# Autodesk Inventor assembly: rovPrototype3
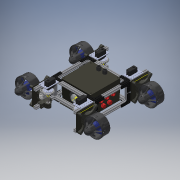
[picture p0: Inventor's stored thumbnail of the model, 180x180]
Saved by Autodesk Inventor 2018 (Build 220112000, 112)
## iProperties
Created: 2019-02-16
Part Number: rovPrototype3
Document SubType Name: Assembly
Designer: anirudh
Author: anirudh
## Documents named in this file (17)
- C:\Users\anirudh\Documents\MARS Fund\MATE Robotics\Silicon Sharks\2018-2019\Prototype3\rovPrototype3.iam
- C:\Users\anirudh\Documents\MARS Fund\MATE Robotics\Silicon Sharks\2018-2019\Prototype3\15inREV(3).ipt
- C:\Users\anirudh\Documents\MARS Fund\MATE Robotics\Silicon Sharks\2018-2019\Prototype3\LazySusanBearing(3).ipt
- C:\Users\anirudh\Documents\MARS Fund\Random CAD Files\REV-41-1305.ipt
- C:\Users\anirudh\Documents\MARS Fund\MATE Robotics\Silicon Sharks\2018-2019\Prototype3\12inREV(3).ipt
- C:\Users\anirudh\Documents\MARS Fund\MATE Robotics\Silicon Sharks\2018-2019\Prototype3\ThrusterMountv2(3).ipt
- C:\Users\anirudh\Documents\MARS Fund\MATE Robotics\Silicon Sharks\2018-2019\Prototype3\BevelGearTest(3).iam
- C:\Users\anirudh\Documents\MARS Fund\Random CAD Files\REV-41-1363.ipt
- C:\Users\anirudh\Documents\MARS Fund\MATE Robotics\Silicon Sharks\2018-2019\Prototype3\Servo(3).ipt
- C:\Users\anirudh\Documents\MARS Fund\Random CAD Files\REV-41-1028.ipt
- C:\Users\anirudh\Documents\MARS Fund\MATE Robotics\Silicon Sharks\2018-2019\Prototype3\4inREV(3).ipt
- C:\Users\anirudh\Documents\MARS Fund\MATE Robotics\Silicon Sharks\2018-2019\Prototype3\T200-THRUSTER(3).ipt
- C:\Users\anirudh\Documents\MARS Fund\MATE Robotics\Silicon Sharks\2018-2019\Prototype3\6mm-2.75inAxle(3).ipt
- C:\Users\anirudh\Documents\MARS Fund\MATE Robotics\Silicon Sharks\2018-2019\Prototype3\AxleBracket(3).ipt
- C:\Users\anirudh\Documents\MARS Fund\Random CAD Files\am-3377 6x12x4 Flanged Bearing.ipt
- C:\Users\anirudh\Documents\MARS Fund\Random CAD Files\REV-41-1480.ipt
- C:\Users\anirudh\Documents\MARS Fund\MATE Robotics\Silicon Sharks\2018-2019\ElectronicsHousing\ElectronicsHousing.iam
## Components (73 placed, 16 different names)
1. 15inREV(3):1 — Flush:1, Flush:2, Flush:4, Mate:3, Mate:4, Flush:11, Flush:12, Mate:21, Mate:22, Flush:13, Flush:14, Mate:137, Flush:69, Flush:71, Mate:172, Mate:173, Flush:86, Mate:184, Mate:185, Flush:89, Flush:94, Mate:196, Flush:96, Flush:99
2. 15inREV(3):2 — Flush:1, Flush:2, Mate:1, Flush:6, Mate:2, Flush:7, Flush:8, Flush:15, Flush:16, Mate:29, Mate:30, Mate:32, Flush:18, Mate:33, Flush:19, Flush:27, Mate:121, Flush:51, Flush:52, Flush:59, Mate:127, Flush:60, Mate:133, Flush:67, Mate:136, Flush:68, Mate:139, Flush:70, Mate:141, Mate:143, Flush:72
3. LazySusanBearing(3):1 — Mate:1, Flush:4, Flush:7, Mate:3, Mate:55, Mate:56, Mate:57, Mate:58, Mate:59, Mate:134
4. LazySusanBearing(3):2 — Flush:6, Mate:2, Flush:8, Mate:4, Mate:60, Mate:61, Mate:62, Mate:63, Mate:64, Mate:135
5. 12inREV(3):1 — Flush:12, Mate:22, Flush:14, Mate:195, Flush:93, Flush:95
6. 12inREV(3):2 — Flush:11, Mate:21, Flush:13, Flush:90, Mate:194, Flush:97, Mate:197, Flush:98, Mate:198
7. 12inREV(3):3 — Flush:16, Mate:30, Mate:32, Flush:20, Mate:34, Flush:26, Mate:40, Flush:31, Mate:42
8. REV-41-1305:7 — Flush:17, Flush:18, Mate:33
9. REV-41-1305:8 — Flush:19, Flush:20, Mate:34
10. 12inREV(3):4 — Flush:15, Mate:29, Flush:17, Flush:29, Mate:41
11. REV-41-1305:10 — Flush:28, Flush:29, Mate:41
12. REV-41-1305:12 — Flush:30, Flush:31, Mate:42
13. 15inREV(3):3 — Flush:24, Flush:25, Mate:39, Flush:26, Mate:40, Flush:27, Flush:28, Flush:30, Mate:120, Flush:48, Flush:49, Flush:65, Mate:132, Mate:145, Flush:73, Mate:147, Flush:74, Mate:149, Mate:151, Flush:76, Mate:153, Mate:155, Flush:78
14. 15inREV(3):4 — Flush:21, Mate:35, Flush:23, Mate:36, Mate:37, Mate:38, Flush:75, Flush:77, Mate:164, Mate:165, Flush:84, Mate:180, Mate:181, Flush:87, Flush:91, Flush:92
15. LazySusanBearing(3):3 — Flush:23, Mate:36, Mate:38, Mate:66, Mate:67, Mate:68, Mate:69, Mate:70, Mate:146
16. LazySusanBearing(3):4 — Flush:21, Mate:35, Mate:37, Flush:24, Flush:25, Mate:39, Mate:65, Mate:71, Mate:72, Mate:73, Mate:74, Mate:148
17. ThrusterMountv2(3):1 — Mate:55, Mate:56, Mate:57, Mate:58, Mate:59, Mate:122, Mate:123, Mate:160
18. ThrusterMountv2(3):2 — Mate:60, Mate:61, Mate:62, Mate:63, Mate:64, Mate:97, Mate:98, Mate:161
19. ThrusterMountv2(3):3 — Mate:65, Mate:71, Mate:72, Mate:73, Mate:74, Mate:103, Mate:159
20. ThrusterMountv2(3):4 — Mate:66, Mate:67, Mate:68, Mate:69, Mate:70, Mate:128, Mate:129, Mate:158
21. BevelGearTest(3):4 [sub-assembly] — Mate:86, Insert:4, Mate:91, Mate:97, Mate:98, Flush:55, Flush:61, Mate:182, Mate:183
22. REV-41-1363:4 — Mate:86, Insert:4, Mate:88
23. Servo(3):4 — Mate:88, Mate:91, Flush:50, Flush:57, Flush:62, Flush:63
24. REV-41-1028:3 — Mate:121, Flush:51, Flush:52, Flush:66
25. BevelGearTest(3):5 [sub-assembly] — Mate:103, Mate:105, Mate:106, Mate:108, Flush:54, Mate:162, Mate:163
26. REV-41-1363:5 — Mate:105, Mate:106, Mate:107
27. Servo(3):5 — Mate:107, Mate:108, Flush:50, Flush:56, Flush:58, Flush:64
28. REV-41-1028:4 — Mate:120, Flush:48, Flush:49
29. BevelGearTest(3):6 [sub-assembly] — Mate:122, Mate:123, Flush:54, Flush:55, Mate:124, Mate:125, Mate:170, Mate:171
30. REV-41-1363:6 — Mate:124, Mate:125, Mate:126
31. Servo(3):6 — Mate:126, Flush:56, Flush:57, Flush:58
32. REV-41-1028:5 — Flush:59, Mate:127, Flush:60
33. Servo(3):7 — Flush:62, Flush:63, Flush:64
34. BevelGearTest(3):7 [sub-assembly] — Mate:128, Flush:61, Mate:129, Mate:130, Mate:131, Mate:157, Mate:178, Mate:179
35. REV-41-1363:7 — Mate:130, Mate:131
36. REV-41-1028:6 — Flush:65, Mate:132, Flush:66
37. REV-41-1305:13 — Mate:139, Flush:70, Mate:140
38. REV-41-1305:14 — Mate:137, Mate:138, Flush:69
39. REV-41-1305:15 — Mate:143, Flush:72, Mate:144
40. REV-41-1305:16 — Mate:141, Flush:71, Mate:142
41. 4inREV(3):1 — Mate:133, Flush:67, Mate:134, Mate:138, Mate:140
42. 4inREV(3):2 — Mate:135, Mate:136, Flush:68, Mate:142, Mate:144
43. 4inREV(3):3 — Mate:145, Flush:73, Mate:146, Mate:150, Mate:152
44. 4inREV(3):4 — Mate:147, Flush:74, Mate:148, Mate:154, Mate:156
45. REV-41-1305:17 — Mate:155, Flush:78, Mate:156
46. REV-41-1305:18 — Mate:153, Flush:77, Mate:154
47. REV-41-1305:19 — Mate:149, Flush:75, Mate:150
48. REV-41-1305:20 — Mate:151, Flush:76, Mate:152
49. T200-THRUSTER(3):1 — Mate:157, Mate:158, Flush:79, Flush:82, Flush:83
50. T200-THRUSTER(3):2 — Mate:159, Flush:79, Flush:80, Flush:81
51. T200-THRUSTER(3):3 — Mate:161, Flush:82, Flush:83
52. T200-THRUSTER(3):4 — Mate:160, Flush:80, Flush:81
53. 6mm-2.75inAxle(3):1 — Mate:162, Mate:163, Mate:168, Mate:169, Flush:85
54. AxleBracket(3):1 — Mate:164, Mate:165, Flush:84, Mate:166, Mate:167
55. am-3377 6x12x4 Flanged Bearing:1 — Mate:167, Mate:168
56. am-3377 6x12x4 Flanged Bearing:2 — Mate:166, Mate:169
57. am-3377 6x12x4 Flanged Bearing:3 — Mate:176, Mate:177
58. am-3377 6x12x4 Flanged Bearing:4 — Mate:174, Mate:175
59. 6mm-2.75inAxle(3):2 — Mate:170, Mate:171, Flush:85, Mate:175, Mate:177
60. AxleBracket(3):2 — Mate:172, Mate:173, Flush:86, Mate:174, Mate:176
61. 6mm-2.75inAxle(3):3 — Mate:178, Mate:179, Flush:88, Mate:191, Mate:193
62. AxleBracket(3):3 — Mate:180, Mate:181, Flush:87, Mate:190, Mate:192
63. 6mm-2.75inAxle(3):4 — Flush:88, Mate:182, Mate:183, Mate:187, Mate:189
64. AxleBracket(3):4 — Mate:184, Mate:185, Flush:89, Mate:186, Mate:188
65. am-3377 6x12x4 Flanged Bearing:5 — Mate:188, Mate:189
66. am-3377 6x12x4 Flanged Bearing:6 — Mate:186, Mate:187
67. am-3377 6x12x4 Flanged Bearing:7 — Mate:190, Mate:191
68. am-3377 6x12x4 Flanged Bearing:8 — Mate:192, Mate:193
69. REV-41-1480:1 — Flush:94, Mate:196, Flush:95
70. REV-41-1480:2 — Flush:90, Flush:91, Mate:194
71. REV-41-1480:3 — Flush:96, Flush:97, Mate:197
72. REV-41-1480:4 — Mate:195, Flush:92, Flush:93
73. ElectronicsHousing:1 [sub-assembly] — Flush:98, Mate:198, Flush:99
## Relationships (206: Mate 128, Flush 77, Insert 1)
- Flush:1: 15inREV(3):1 ↔ 15inREV(3):2
- Flush:2: 15inREV(3):1 ↔ 15inREV(3):2
- Mate:1: 15inREV(3):2 ↔ LazySusanBearing(3):1
- Flush:4: 15inREV(3):1 ↔ LazySusanBearing(3):1
- Flush:6: 15inREV(3):2 ↔ LazySusanBearing(3):2
- Mate:2: 15inREV(3):2 ↔ LazySusanBearing(3):2
- Flush:7: 15inREV(3):2 ↔ LazySusanBearing(3):1
- Mate:3: 15inREV(3):1 ↔ LazySusanBearing(3):1
- Flush:8: 15inREV(3):2 ↔ LazySusanBearing(3):2
- Mate:4: 15inREV(3):1 ↔ LazySusanBearing(3):2
- Flush:11: 15inREV(3):1 ↔ 12inREV(3):2
- Flush:12: 15inREV(3):1 ↔ 12inREV(3):1
- Mate:21: 15inREV(3):1 ↔ 12inREV(3):2
- Mate:22: 15inREV(3):1 ↔ 12inREV(3):1
- Flush:13 (97.2693 mm): 15inREV(3):1 ↔ 12inREV(3):2
- Flush:14 (97.2693 mm): 15inREV(3):1 ↔ 12inREV(3):1
- Flush:15: 15inREV(3):2 ↔ 12inREV(3):4
- Flush:16: 15inREV(3):2 ↔ 12inREV(3):3
- Mate:29: 15inREV(3):2 ↔ 12inREV(3):4
- Mate:30: 15inREV(3):2 ↔ 12inREV(3):3
- Mate:32 (-108.712 mm): 15inREV(3):2 ↔ 12inREV(3):3
- Flush:17: REV-41-1305:7 ↔ 12inREV(3):4
- Flush:18: 15inREV(3):2 ↔ REV-41-1305:7
- Mate:33: 15inREV(3):2 ↔ REV-41-1305:7
- Flush:19: 15inREV(3):2 ↔ REV-41-1305:8
- Flush:20: 12inREV(3):3 ↔ REV-41-1305:8
- Mate:34: 12inREV(3):3 ↔ REV-41-1305:8
- Flush:21: 15inREV(3):4 ↔ LazySusanBearing(3):4
- Mate:35: 15inREV(3):4 ↔ LazySusanBearing(3):4
- Flush:23: 15inREV(3):4 ↔ LazySusanBearing(3):3
- Mate:36: 15inREV(3):4 ↔ LazySusanBearing(3):3
- Mate:37: 15inREV(3):4 ↔ LazySusanBearing(3):4
- Mate:38: 15inREV(3):4 ↔ LazySusanBearing(3):3
- Flush:24: 15inREV(3):3 ↔ LazySusanBearing(3):4
- Flush:25: 15inREV(3):3 ↔ LazySusanBearing(3):4
- Mate:39: 15inREV(3):3 ↔ LazySusanBearing(3):4
- Flush:26: 12inREV(3):3 ↔ 15inREV(3):3
- Mate:40: 12inREV(3):3 ↔ 15inREV(3):3
- Flush:27: 15inREV(3):2 ↔ 15inREV(3):3
- Flush:28: REV-41-1305:10 ↔ 15inREV(3):3
- Flush:29: 12inREV(3):4 ↔ REV-41-1305:10
- Mate:41: 12inREV(3):4 ↔ REV-41-1305:10
- Flush:30: REV-41-1305:12 ↔ 15inREV(3):3
- Flush:31: 12inREV(3):3 ↔ REV-41-1305:12
- Mate:42: 12inREV(3):3 ↔ REV-41-1305:12
- Mate:55: LazySusanBearing(3):1 ↔ ThrusterMountv2(3):1
- Mate:56: LazySusanBearing(3):1 ↔ ThrusterMountv2(3):1
- Mate:57: LazySusanBearing(3):1 ↔ ThrusterMountv2(3):1
- Mate:58: LazySusanBearing(3):1 ↔ ThrusterMountv2(3):1
- Mate:59: LazySusanBearing(3):1 ↔ ThrusterMountv2(3):1
- Mate:60: LazySusanBearing(3):2 ↔ ThrusterMountv2(3):2
- Mate:61: LazySusanBearing(3):2 ↔ ThrusterMountv2(3):2
- Mate:62: LazySusanBearing(3):2 ↔ ThrusterMountv2(3):2
- Mate:63: LazySusanBearing(3):2 ↔ ThrusterMountv2(3):2
- Mate:64: LazySusanBearing(3):2 ↔ ThrusterMountv2(3):2
- Mate:65: LazySusanBearing(3):4 ↔ ThrusterMountv2(3):3
- Mate:66: LazySusanBearing(3):3 ↔ ThrusterMountv2(3):4
- Mate:67: LazySusanBearing(3):3 ↔ ThrusterMountv2(3):4
- Mate:68: LazySusanBearing(3):3 ↔ ThrusterMountv2(3):4
- Mate:69: LazySusanBearing(3):3 ↔ ThrusterMountv2(3):4
- Mate:70: LazySusanBearing(3):3 ↔ ThrusterMountv2(3):4
- Mate:71: LazySusanBearing(3):4 ↔ ThrusterMountv2(3):3
- Mate:72: LazySusanBearing(3):4 ↔ ThrusterMountv2(3):3
- Mate:73: LazySusanBearing(3):4 ↔ ThrusterMountv2(3):3
- Mate:74: LazySusanBearing(3):4 ↔ ThrusterMountv2(3):3
- Mate:86: BevelGearTest(3):4 ↔ REV-41-1363:4
- Insert:4: BevelGearTest(3):4 ↔ REV-41-1363:4
- Mate:88: REV-41-1363:4 ↔ Servo(3):4
- Mate:91: BevelGearTest(3):4 ↔ Servo(3):4
- Mate:97: ThrusterMountv2(3):2 ↔ BevelGearTest(3):4
- Mate:98: ThrusterMountv2(3):2 ↔ BevelGearTest(3):4
- Mate:103: ThrusterMountv2(3):3 ↔ BevelGearTest(3):5
- Mate:105: BevelGearTest(3):5 ↔ REV-41-1363:5
- Mate:106: BevelGearTest(3):5 ↔ REV-41-1363:5
- Mate:107: REV-41-1363:5 ↔ Servo(3):5
- Mate:108: BevelGearTest(3):5 ↔ Servo(3):5
- Mate:120: 15inREV(3):3 ↔ REV-41-1028:4
- Flush:48: 15inREV(3):3 ↔ REV-41-1028:4
- Flush:49 (25.1206 mm): 15inREV(3):3 ↔ REV-41-1028:4
- Flush:50: Servo(3):4 ↔ Servo(3):5
- Mate:121: 15inREV(3):2 ↔ REV-41-1028:3
- Flush:51: 15inREV(3):2 ↔ REV-41-1028:3
- Flush:52 (25.1206 mm): 15inREV(3):2 ↔ REV-41-1028:3
- Mate:122: ThrusterMountv2(3):1 ↔ BevelGearTest(3):6
- Mate:123: ThrusterMountv2(3):1 ↔ BevelGearTest(3):6
- Flush:54: BevelGearTest(3):5 ↔ BevelGearTest(3):6
- Flush:55: BevelGearTest(3):4 ↔ BevelGearTest(3):6
- Mate:124: BevelGearTest(3):6 ↔ REV-41-1363:6
- Mate:125: BevelGearTest(3):6 ↔ REV-41-1363:6
- Mate:126: REV-41-1363:6 ↔ Servo(3):6
- Flush:56: Servo(3):5 ↔ Servo(3):6
- Flush:57: Servo(3):4 ↔ Servo(3):6
- Flush:58: Servo(3):5 ↔ Servo(3):6
- Flush:59: 15inREV(3):2 ↔ REV-41-1028:5
- Mate:127: 15inREV(3):2 ↔ REV-41-1028:5
- Flush:60 (25.1206 mm): 15inREV(3):2 ↔ REV-41-1028:5
- Mate:128: ThrusterMountv2(3):4 ↔ BevelGearTest(3):7
- Flush:61: BevelGearTest(3):4 ↔ BevelGearTest(3):7
- Mate:129: ThrusterMountv2(3):4 ↔ BevelGearTest(3):7
- Mate:130: BevelGearTest(3):7 ↔ REV-41-1363:7
- Mate:131: BevelGearTest(3):7 ↔ REV-41-1363:7
- Flush:62: Servo(3):4 ↔ Servo(3):7
- Flush:63: Servo(3):4 ↔ Servo(3):7
- Flush:64: Servo(3):5 ↔ Servo(3):7
- Flush:65: 15inREV(3):3 ↔ REV-41-1028:6
- Mate:132: 15inREV(3):3 ↔ REV-41-1028:6
- Flush:66: REV-41-1028:3 ↔ REV-41-1028:6
- Mate:133: 15inREV(3):2 ↔ 4inREV(3):1
- Flush:67: 15inREV(3):2 ↔ 4inREV(3):1
- Mate:134 (2.54 mm): LazySusanBearing(3):1 ↔ 4inREV(3):1
- Mate:135 (2.54 mm): LazySusanBearing(3):2 ↔ 4inREV(3):2
- Mate:136: 15inREV(3):2 ↔ 4inREV(3):2
- Flush:68: 15inREV(3):2 ↔ 4inREV(3):2
- Mate:137: 15inREV(3):1 ↔ REV-41-1305:14
- Mate:138: REV-41-1305:14 ↔ 4inREV(3):1
- Flush:69: 15inREV(3):1 ↔ REV-41-1305:14
- Mate:139: 15inREV(3):2 ↔ REV-41-1305:13
- Flush:70: 15inREV(3):2 ↔ REV-41-1305:13
- Mate:140: REV-41-1305:13 ↔ 4inREV(3):1
- Mate:141: 15inREV(3):2 ↔ REV-41-1305:16
- Flush:71: 15inREV(3):1 ↔ REV-41-1305:16
- Mate:142: REV-41-1305:16 ↔ 4inREV(3):2
- Mate:143: 15inREV(3):2 ↔ REV-41-1305:15
- Flush:72: 15inREV(3):2 ↔ REV-41-1305:15
- Mate:144: REV-41-1305:15 ↔ 4inREV(3):2
- Mate:145: 15inREV(3):3 ↔ 4inREV(3):3
- Flush:73: 15inREV(3):3 ↔ 4inREV(3):3
- Mate:146 (2.54 mm): LazySusanBearing(3):3 ↔ 4inREV(3):3
- Mate:147: 15inREV(3):3 ↔ 4inREV(3):4
- Flush:74: 15inREV(3):3 ↔ 4inREV(3):4
- Mate:148 (2.54 mm): LazySusanBearing(3):4 ↔ 4inREV(3):4
- Mate:149: 15inREV(3):3 ↔ REV-41-1305:19
- Flush:75: 15inREV(3):4 ↔ REV-41-1305:19
- Mate:150: 4inREV(3):3 ↔ REV-41-1305:19
- Mate:151: 15inREV(3):3 ↔ REV-41-1305:20
- Flush:76: 15inREV(3):3 ↔ REV-41-1305:20
- Mate:152: 4inREV(3):3 ↔ REV-41-1305:20
- Mate:153: 15inREV(3):3 ↔ REV-41-1305:18
- Flush:77: 15inREV(3):4 ↔ REV-41-1305:18
- Mate:154: 4inREV(3):4 ↔ REV-41-1305:18
- Mate:155: 15inREV(3):3 ↔ REV-41-1305:17
- Flush:78: 15inREV(3):3 ↔ REV-41-1305:17
- Mate:156: 4inREV(3):4 ↔ REV-41-1305:17
- Mate:157: BevelGearTest(3):7 ↔ T200-THRUSTER(3):1
- Mate:158: ThrusterMountv2(3):4 ↔ T200-THRUSTER(3):1
- Mate:159: ThrusterMountv2(3):3 ↔ T200-THRUSTER(3):2
- Flush:79: T200-THRUSTER(3):1 ↔ T200-THRUSTER(3):2
- Mate:160: ThrusterMountv2(3):1 ↔ T200-THRUSTER(3):4
- Flush:80: T200-THRUSTER(3):2 ↔ T200-THRUSTER(3):4
- Flush:81: T200-THRUSTER(3):2 ↔ T200-THRUSTER(3):4
- Mate:161: ThrusterMountv2(3):2 ↔ T200-THRUSTER(3):3
- Flush:82: T200-THRUSTER(3):1 ↔ T200-THRUSTER(3):3
- Flush:83: T200-THRUSTER(3):1 ↔ T200-THRUSTER(3):3
- Mate:162 (-6.35 mm): BevelGearTest(3):5 ↔ 6mm-2.75inAxle(3):1
- Mate:163: BevelGearTest(3):5 ↔ 6mm-2.75inAxle(3):1
- Mate:164: 15inREV(3):4 ↔ AxleBracket(3):1
- Mate:165: 15inREV(3):4 ↔ AxleBracket(3):1
- Flush:84 (19.9136 mm): 15inREV(3):4 ↔ AxleBracket(3):1
- Mate:166: AxleBracket(3):1 ↔ am-3377 6x12x4 Flanged Bearing:2
- Mate:167: AxleBracket(3):1 ↔ am-3377 6x12x4 Flanged Bearing:1
- Mate:168: 6mm-2.75inAxle(3):1 ↔ am-3377 6x12x4 Flanged Bearing:1
- Mate:169: 6mm-2.75inAxle(3):1 ↔ am-3377 6x12x4 Flanged Bearing:2
- Mate:170 (-6.35 mm): BevelGearTest(3):6 ↔ 6mm-2.75inAxle(3):2
- Mate:171: BevelGearTest(3):6 ↔ 6mm-2.75inAxle(3):2
- Flush:85: 6mm-2.75inAxle(3):1 ↔ 6mm-2.75inAxle(3):2
- Mate:172: 15inREV(3):1 ↔ AxleBracket(3):2
- Mate:173: 15inREV(3):1 ↔ AxleBracket(3):2
- Flush:86 (19.9136 mm): 15inREV(3):1 ↔ AxleBracket(3):2
- Mate:174: am-3377 6x12x4 Flanged Bearing:4 ↔ AxleBracket(3):2
- Mate:175: am-3377 6x12x4 Flanged Bearing:4 ↔ 6mm-2.75inAxle(3):2
- Mate:176: am-3377 6x12x4 Flanged Bearing:3 ↔ AxleBracket(3):2
- Mate:177: am-3377 6x12x4 Flanged Bearing:3 ↔ 6mm-2.75inAxle(3):2
- Mate:178 (-6.35 mm): BevelGearTest(3):7 ↔ 6mm-2.75inAxle(3):3
- Mate:179: BevelGearTest(3):7 ↔ 6mm-2.75inAxle(3):3
- Mate:180: 15inREV(3):4 ↔ AxleBracket(3):3
- Mate:181: 15inREV(3):4 ↔ AxleBracket(3):3
- Flush:87 (19.9136 mm): 15inREV(3):4 ↔ AxleBracket(3):3
- Flush:88: 6mm-2.75inAxle(3):3 ↔ 6mm-2.75inAxle(3):4
- Mate:182: BevelGearTest(3):4 ↔ 6mm-2.75inAxle(3):4
- Mate:183 (-6.35 mm): BevelGearTest(3):4 ↔ 6mm-2.75inAxle(3):4
- Mate:184: 15inREV(3):1 ↔ AxleBracket(3):4
- Mate:185: 15inREV(3):1 ↔ AxleBracket(3):4
- Flush:89 (19.9136 mm): 15inREV(3):1 ↔ AxleBracket(3):4
- Mate:186: AxleBracket(3):4 ↔ am-3377 6x12x4 Flanged Bearing:6
- Mate:187: 6mm-2.75inAxle(3):4 ↔ am-3377 6x12x4 Flanged Bearing:6
- Mate:188: AxleBracket(3):4 ↔ am-3377 6x12x4 Flanged Bearing:5
- Mate:189: 6mm-2.75inAxle(3):4 ↔ am-3377 6x12x4 Flanged Bearing:5
- Mate:190: AxleBracket(3):3 ↔ am-3377 6x12x4 Flanged Bearing:7
- Mate:191: 6mm-2.75inAxle(3):3 ↔ am-3377 6x12x4 Flanged Bearing:7
- Mate:192: AxleBracket(3):3 ↔ am-3377 6x12x4 Flanged Bearing:8
- Mate:193: 6mm-2.75inAxle(3):3 ↔ am-3377 6x12x4 Flanged Bearing:8
- Flush:90: 12inREV(3):2 ↔ REV-41-1480:2
- Flush:91: 15inREV(3):4 ↔ REV-41-1480:2
- Mate:194: 12inREV(3):2 ↔ REV-41-1480:2
- Mate:195: 12inREV(3):1 ↔ REV-41-1480:4
- Flush:92: 15inREV(3):4 ↔ REV-41-1480:4
- Flush:93: 12inREV(3):1 ↔ REV-41-1480:4
- Flush:94: 15inREV(3):1 ↔ REV-41-1480:1
- Mate:196: 15inREV(3):1 ↔ REV-41-1480:1
- Flush:95: 12inREV(3):1 ↔ REV-41-1480:1
- Flush:96: 15inREV(3):1 ↔ REV-41-1480:3
- Flush:97: 12inREV(3):2 ↔ REV-41-1480:3
- Mate:197: 12inREV(3):2 ↔ REV-41-1480:3
- Flush:98 (-0.4191 mm): 12inREV(3):2 ↔ ElectronicsHousing:1
- Mate:198: 12inREV(3):2 ↔ ElectronicsHousing:1
- Flush:99 (38.0238 mm): 15inREV(3):1 ↔ ElectronicsHousing:1
